# Autodesk Inventor assembly: Assembly.
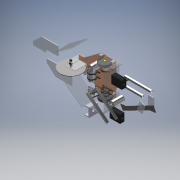
[picture p0: Inventor's stored thumbnail of the model, 180x180]
Saved by Autodesk Inventor 2019 (Build 230136000, 136)
## iProperties
Created: 2018-08-16
Part Number: Assembly.
Document SubType Name: Assembly
Designer: andres2416
Author: andres2416
## Documents named in this file (26)
- C:\Users\garstka1245\Downloads\bot\full-bot-assembly.iam
- C:\Users\garstka1245\Downloads\bot\Electronics\battery.ipt
- C:\Users\garstka1245\Downloads\bot\Motor Mount H\motor-mount-h-E30-bot.ipt
- C:\Users\garstka1245\Downloads\bot\Motor Mount H\motor-mount-h-E30-top.ipt
- C:\Users\garstka1245\Downloads\bot\Mechanicals\motor-E30-400.ipt
- C:\Users\garstka1245\Downloads\bot\Structure\bar-aluminium.ipt
- C:\Users\garstka1245\Downloads\bot\Structure\standoff.ipt
- C:\Users\garstka1245\Downloads\bot\Weapon Saw\wall-side-saw.ipt
- C:\Users\garstka1245\Downloads\bot\Weapon Saw\wall-saw-support.ipt
- C:\Users\garstka1245\Downloads\bot\Weapon Saw\wall-side-saw-hole.ipt
- C:\Users\garstka1245\Downloads\bot\Weapon Saw\weapon-saw.ipt
- C:\Users\garstka1245\Downloads\bot\Mechanicals\wheel-6in.ipt
- C:\Users\garstka1245\Downloads\bot\Weapon Saw\axle-saw.ipt
- C:\Users\garstka1245\Downloads\bot\Shell\base\base.ipt
- C:\Users\garstka1245\Downloads\bot\Shell\second-layer\platform.ipt
- C:\Users\garstka1245\Downloads\bot\Mechanicals\gear-vex.ipt
- C:\Users\garstka1245\Downloads\bot\Weapon Saw\axle-shaft-collar-saw.ipt
- C:\Users\garstka1245\Downloads\bot\Weapon Spinner\mount-point.ipt
- C:\Users\garstka1245\Downloads\bot\Weapon Spinner\axle-spinner.ipt
- C:\Users\garstka1245\Downloads\bot\Weapon Spinner\weapon-spinner.ipt
- C:\Users\garstka1245\Downloads\bot\Shell\wall-parts\wall-spinner.ipt
- C:\Users\garstka1245\Downloads\bot\Shell\wall-parts\wall-side.ipt
- C:\Users\garstka1245\Downloads\bot\Shell\wall-parts\wall-angled.ipt
- C:\Users\garstka1245\Downloads\bot\Structure\bracket-aluminium.ipt
- C:\Users\garstka1245\Downloads\bot\Motor Mount V\motor-mount-v-E30.ipt
- C:\Users\garstka1245\Downloads\bot\Mechanicals\pillowblock.ipt
## Components (61 placed, 25 different names)
1. battery:1
2. battery:3
3. wheel-6in:2
4. wheel-6in:1
5. gear-vex:1
6. gear-vex:2
7. pillowblock:1
8. pillowblock:2
9. motor-E30-400:1
10. motor-E30-400:2
11. motor-E30-400:3 — Mate:21, Mate:23
12. motor-mount-h-E30-bot:1
13. motor-mount-h-E30-bot:2
14. motor-mount-h-E30-top:2
15. motor-mount-h-E30-bot:3
16. motor-mount-h-E30-top:3
17. motor-mount-h-E30-bot:4
18. motor-mount-h-E30-bot:5 — Mate:23, Mate:24, Mate:25, Mate:27
19. motor-mount-h-E30-top:7 — Mate:25, Mate:27
20. motor-mount-h-E30-bot:6 — Mate:21, Mate:22, Mate:26, Mate:28
21. motor-mount-h-E30-top:8 — Mate:26, Mate:28
22. motor-mount-h-E30-top:5
23. motor-mount-h-E30-top:6
24. motor-mount-v-E30:1
25. platform:2
26. platform:1
27. base:1 — Mate:1, Mate:2, Mate:3, Mate:4, Mate:5, Mate:6, Mate:7, Mate:8, Mate:9, Mate:10, Mate:11, Mate:12, Mate:13, Mate:14, Mate:15, Mate:16, Mate:17, Mate:18, Mate:19, Mate:22, Mate:24
28. wall-side:1
29. wall-side:2
30. wall-spinner:1
31. wall-angled:2
32. wall-angled:1
33. standoff:4 — Mate:29, Mate:35, Mate:38, Mate:39
34. standoff:3 — Mate:31, Mate:33
35. standoff:2 — Mate:36, Mate:43
36. standoff:1 — Mate:37, Mate:40, Mate:41, Mate:42
37. bar-aluminium:1 — Mate:33, Mate:35, Mate:38
38. bar-aluminium:2 — Mate:36, Mate:37, Mate:40
39. bar-aluminium:3 — Mate:29, Mate:31, Mate:39
40. bar-aluminium:4 — Mate:41, Mate:42, Mate:43
41. bracket-aluminium:1 — Mate:15
42. bracket-aluminium:2 — Mate:12, Mate:16
43. bracket-aluminium:3 — Mate:11, Mate:14
44. bracket-aluminium:4 — Mate:6, Mate:8
45. bracket-aluminium:5 — Mate:9, Mate:19
46. bracket-aluminium:6 — Mate:1, Mate:2
47. bracket-aluminium:7 — Mate:10, Mate:18
48. bracket-aluminium:8 — Mate:13, Mate:17
49. bracket-aluminium:9 — Mate:3, Mate:4
50. bracket-aluminium:10 — Mate:5, Mate:7
51. wall-side-saw-hole:1
52. wall-saw-support:1
53. wall-side-saw:1
54. weapon-saw:1
55. axle-saw:1
56. axle-shaft-collar-saw:1
57. axle-shaft-collar-saw:2
58. mount-point:1
59. mount-point:2
60. axle-spinner:1 — Mate:20, Flush:1
61. weapon-spinner:1 — Mate:20, Flush:1
## Relationships (41: Mate 40, Flush 1)
- Mate:1: base:1 ↔ bracket-aluminium:6
- Mate:2: base:1 ↔ bracket-aluminium:6
- Mate:3: base:1 ↔ bracket-aluminium:9
- Mate:4: base:1 ↔ bracket-aluminium:9
- Mate:5: base:1 ↔ bracket-aluminium:10
- Mate:6: base:1 ↔ bracket-aluminium:4
- Mate:7: base:1 ↔ bracket-aluminium:10
- Mate:8: base:1 ↔ bracket-aluminium:4
- Mate:9: base:1 ↔ bracket-aluminium:5
- Mate:10: base:1 ↔ bracket-aluminium:7
- Mate:11: base:1 ↔ bracket-aluminium:3
- Mate:12: base:1 ↔ bracket-aluminium:2
- Mate:13: base:1 ↔ bracket-aluminium:8
- Mate:14: base:1 ↔ bracket-aluminium:3
- Mate:15: base:1 ↔ bracket-aluminium:1
- Mate:16: base:1 ↔ bracket-aluminium:2
- Mate:17: base:1 ↔ bracket-aluminium:8
- Mate:18: base:1 ↔ bracket-aluminium:7
- Mate:19: base:1 ↔ bracket-aluminium:5
- Mate:20: axle-spinner:1 ↔ weapon-spinner:1
- Flush:1 (50.8 mm): axle-spinner:1 ↔ weapon-spinner:1
- Mate:21: motor-E30-400:3 ↔ motor-mount-h-E30-bot:6
- Mate:22: motor-mount-h-E30-bot:6 ↔ base:1
- Mate:23: motor-E30-400:3 ↔ motor-mount-h-E30-bot:5
- Mate:24: motor-mount-h-E30-bot:5 ↔ base:1
- Mate:25: motor-mount-h-E30-bot:5 ↔ motor-mount-h-E30-top:7
- Mate:26: motor-mount-h-E30-bot:6 ↔ motor-mount-h-E30-top:8
- Mate:27: motor-mount-h-E30-bot:5 ↔ motor-mount-h-E30-top:7
- Mate:28: motor-mount-h-E30-bot:6 ↔ motor-mount-h-E30-top:8
- Mate:29: standoff:4 ↔ bar-aluminium:3
- Mate:31: standoff:3 ↔ bar-aluminium:3
- Mate:33: standoff:3 ↔ bar-aluminium:1
- Mate:35: standoff:4 ↔ bar-aluminium:1
- Mate:36: standoff:2 ↔ bar-aluminium:2
- Mate:37: standoff:1 ↔ bar-aluminium:2
- Mate:38: standoff:4 ↔ bar-aluminium:1
- Mate:39: standoff:4 ↔ bar-aluminium:3
- Mate:40: standoff:1 ↔ bar-aluminium:2
- Mate:41: standoff:1 ↔ bar-aluminium:4
- Mate:42: standoff:1 ↔ bar-aluminium:4
- Mate:43: standoff:2 ↔ bar-aluminium:4
